# Autodesk Inventor assembly: Build Plate
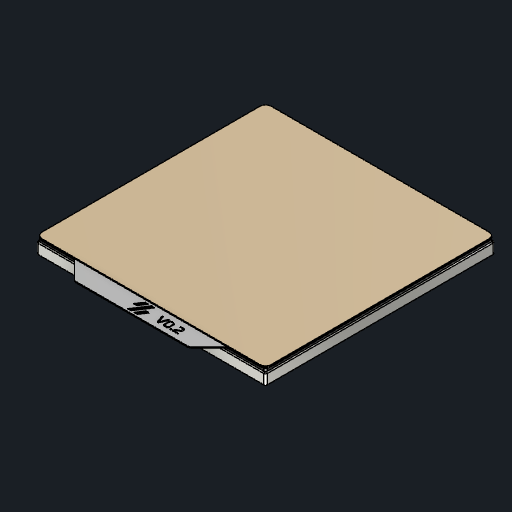
[picture p0: Inventor's stored thumbnail of the model, 512x512]
Saved by Autodesk Inventor 2026.1 (Build 301233020, 233B)
## iProperties
Created: 2025-05-09
Part Number: Build Plate
Document SubType Name: Assembly
Designer: AdminForWorker
Title: Build Plate
Author: AdminForWorker
## Documents named in this file (5)
- C:\Users\JoshuaEah\Documents\GitHub\Voron-0\CAD\Z Axis\Subassemblies\Build Plate.iam
- C:\Users\JoshuaEah\Documents\GitHub\Voron-0\CAD\Z Axis\Parts\120x120mm MIC6.ipt
- C:\Users\JoshuaEah\Documents\GitHub\Voron-0\CAD\Z Axis\Parts\100x100mm Silicone Bed Heater.ipt
- C:\Users\JoshuaEah\Documents\GitHub\Voron-0\CAD\Z Axis\Parts\Magnetic Sheet.ipt
- C:\Users\JoshuaEah\Documents\GitHub\Voron-0\CAD\Z Axis\Parts\Flex Plate.ipt
## Components (4 placed, 4 different names)
1. 120x120mm MIC6:1 — Insert:1, Insert:2
2. 100x100mm Silicone Bed Heater:1
3. Magnetic Sheet:1 — Insert:1, Insert:2, Mate:1, Flush:1, Flush:2
4. Flex Plate:1 — Mate:1, Flush:1, Flush:2
## Relationships (5: Insert 2, Flush 2, Mate 1)
- Insert:1: 120x120mm MIC6:1 ↔ Magnetic Sheet:1
- Insert:2: 120x120mm MIC6:1 ↔ Magnetic Sheet:1
- Mate:1: Magnetic Sheet:1 ↔ Flex Plate:1
- Flush:1 (-0.5 mm): Magnetic Sheet:1 ↔ Flex Plate:1
- Flush:2 (-0.5 mm): Magnetic Sheet:1 ↔ Flex Plate:1
